# Autodesk Inventor assembly: GPS_module
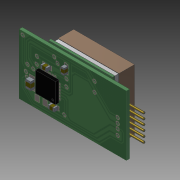
[picture p0: Inventor's stored thumbnail of the model, 180x180]
Saved by Autodesk Inventor 2013 (Build 170138000, 138)
## iProperties
Created: 2015-07-02
Part Number: GPS_module
Document SubType Name: Assembly
Designer: terg
Author: terg
## Documents named in this file (9)
- C:\Users\terg\Projects\ModularElectronics\3D_models\GPS_module\GPS_module.iam
- C:\Users\terg\Projects\ModularElectronics\3D_models\GPS_module\GPS_module_PCB.ipt
- C:\Users\terg\Projects\ModularElectronics\3D_models\Components\0805_cap.ipt
- C:\Users\terg\Projects\ModularElectronics\3D_models\Components\0603_cap.ipt
- C:\Users\terg\Projects\ModularElectronics\3D_models\Components\0805_res.ipt
- C:\Users\terg\Projects\ModularElectronics\3D_models\Components\EFM32ZG110.ipt
- C:\Users\terg\Projects\ModularElectronics\3D_models\GPS_module\FGPMMOPA6C.ipt
- C:\Users\terg\Projects\ModularElectronics\3D_models\Components\FemalConnector.ipt
- C:\Users\terg\Projects\ModularElectronics\3D_models\Components\MaleConnector.ipt
## Components (14 placed, 8 different names)
1. GPS_module_PCB:1 — Zestawiający:1, Zestawiający:2, Zestawiający:3, Zestawiający:4, Zestawiający:5, Zestawiający:6, Zestawiający:7, Zestawiający:8, Równoległy:1, Równoległy:2, Zestawiający:9, Równoległy:3, Równoległy:4, Zestawiający:10, Równoległy:5, Równoległy:6, Zestawiający:11, Równoległy:7, Równoległy:8, Zestawiający:12, Zestawiający:13, Równoległy:9, Równoległy:10, Równoległy:11, Równoległy:12
2. 0805_cap:1 — Zestawiający:1
3. 0805_cap:2 — Zestawiający:3
4. 0603_cap:1 — Zestawiający:2
5. 0805_cap:3 — Zestawiający:4
6. 0603_cap:2 — Zestawiający:5
7. 0603_cap:3 — Zestawiający:6
8. 0603_cap:4 — Zestawiający:7
9. 0805_res:1 — Zestawiający:8, Równoległy:1, Równoległy:2
10. 0603_cap:5 — Zestawiający:9, Równoległy:3, Równoległy:4
11. EFM32ZG110:1 — Zestawiający:10, Równoległy:5, Równoległy:6
12. FGPMMOPA6C:1 — Zestawiający:11, Równoległy:7, Równoległy:8
13. FemalConnector:1 — Zestawiający:12, Równoległy:11, Równoległy:12
14. MaleConnector:1 — Zestawiający:13, Równoległy:9, Równoległy:10
## Relationships (25: Mate 13, Flush 12)
- Zestawiający:1 [Mate]: GPS_module_PCB:1 ↔ 0805_cap:1
- Zestawiający:2 [Mate]: GPS_module_PCB:1 ↔ 0603_cap:1
- Zestawiający:3 [Mate]: GPS_module_PCB:1 ↔ 0805_cap:2
- Zestawiający:4 [Mate]: GPS_module_PCB:1 ↔ 0805_cap:3
- Zestawiający:5 [Mate]: GPS_module_PCB:1 ↔ 0603_cap:2
- Zestawiający:6 [Mate]: GPS_module_PCB:1 ↔ 0603_cap:3
- Zestawiający:7 [Mate]: GPS_module_PCB:1 ↔ 0603_cap:4
- Zestawiający:8 [Mate]: GPS_module_PCB:1 ↔ 0805_res:1
- Równoległy:1 [Flush] (0.618 mm): GPS_module_PCB:1 ↔ 0805_res:1
- Równoległy:2 [Flush] (0.943 mm): GPS_module_PCB:1 ↔ 0805_res:1
- Zestawiający:9 [Mate]: GPS_module_PCB:1 ↔ 0603_cap:5
- Równoległy:3 [Flush] (0.931 mm): GPS_module_PCB:1 ↔ 0603_cap:5
- Równoległy:4 [Flush] (1.692 mm): GPS_module_PCB:1 ↔ 0603_cap:5
- Zestawiający:10 [Mate]: GPS_module_PCB:1 ↔ EFM32ZG110:1
- Równoległy:5 [Flush] (4.03 mm): GPS_module_PCB:1 ↔ EFM32ZG110:1
- Równoległy:6 [Flush] (4.92 mm): GPS_module_PCB:1 ↔ EFM32ZG110:1
- Zestawiający:11 [Mate]: GPS_module_PCB:1 ↔ FGPMMOPA6C:1
- Równoległy:7 [Flush] (4.251 mm): GPS_module_PCB:1 ↔ FGPMMOPA6C:1
- Równoległy:8 [Flush] (-0.46 mm): GPS_module_PCB:1 ↔ FGPMMOPA6C:1
- Zestawiający:12 [Mate]: GPS_module_PCB:1 ↔ FemalConnector:1
- Zestawiający:13 [Mate]: GPS_module_PCB:1 ↔ MaleConnector:1
- Równoległy:9 [Flush] (4.154 mm): GPS_module_PCB:1 ↔ MaleConnector:1
- Równoległy:10 [Flush] (2.87 mm): GPS_module_PCB:1 ↔ MaleConnector:1
- Równoległy:11 [Flush] (3.65 mm): GPS_module_PCB:1 ↔ FemalConnector:1
- Równoległy:12 [Flush] (-0.712 mm): GPS_module_PCB:1 ↔ FemalConnector:1
